# Autodesk Inventor assembly: 01.02.03.00 - Braço esquerdo
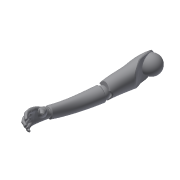
[picture p0: Inventor's stored thumbnail of the model, 180x180]
Saved by Autodesk Inventor 2016 (Build 200138000, 138)
## iProperties
Created: 2017-03-23
Part Number: 01.02.03.00 - Braço esquerdo
Document SubType Name: Assembly
Designer: Wesley Perez
Author: Wesley Perez
## Documents named in this file (4)
- D:\EMPRESARIAL\ADEBOTT\Dep. PROJETOS\ADEBOTT - KIT PROJETISTA\Corpos Humanos\Corpo Humano 01\Parts\01.02.02.00 - Braço direito.iam
- D:\EMPRESARIAL\ADEBOTT\Dep. PROJETOS\ADEBOTT - KIT PROJETISTA\Corpos Humanos\Corpo Humano 01\Parts\01.02.02.01 - Braço direito.ipt
- D:\EMPRESARIAL\ADEBOTT\Dep. PROJETOS\ADEBOTT - KIT PROJETISTA\Corpos Humanos\Corpo Humano 01\Parts\01.02.02.02 - Antebraço direito.ipt
- D:\EMPRESARIAL\ADEBOTT\Dep. PROJETOS\ADEBOTT - KIT PROJETISTA\Corpos Humanos\Corpo Humano 01\Parts\01.02.02.03 - Mão direita.ipt
## Components (3 placed, 3 different names)
1. 01.02.02.01 - Braço direito:1 — Alinhamento:3, Alinhamento:4, Alinhamento:5, Coincidência:1
2. 01.02.02.02 - Antebraço direito:1 — Coincidência:1, Coincidência:2
3. 01.02.02.03 - Mão direita:1 — Coincidência:2
## Relationships (5: Flush 3, Mate 2)
- Alinhamento:3 [Flush]: 01.02.02.01 - Braço direito:1
- Alinhamento:4 [Flush]: 01.02.02.01 - Braço direito:1
- Alinhamento:5 [Flush]: 01.02.02.01 - Braço direito:1
- Coincidência:1 [Mate]: 01.02.02.01 - Braço direito:1 ↔ 01.02.02.02 - Antebraço direito:1
- Coincidência:2 [Mate]: 01.02.02.02 - Antebraço direito:1 ↔ 01.02.02.03 - Mão direita:1
